# Autodesk Inventor assembly: Übertragung des Zahnriemens
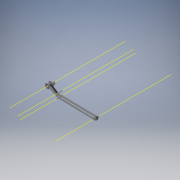
[picture p0: Inventor's stored thumbnail of the model, 180x180]
Saved by Autodesk Inventor 2019.1 (Build 231200000, 200)
## iProperties
Created: 2018-11-28
Part Number: Übertragung des Zahnriemens
Document SubType Name: Assembly
Designer: JochenAlt
ClientObjectVersion: 1
Author: JochenAlt
## Documents named in this file (6)
- D:\Projects\Ondine\CAD\Leg\LegInnerGear\Übertragung des Zahnriemens1.iam
- D:\Projects\Ondine\CAD\Leg\LegInnerGear\Zahnriemen1.ipt
- D:\Projects\Ondine\CAD\Leg\LegInnerGear\Synchrone Riemenscheibe11.ipt
- D:\Projects\Ondine\CAD\Leg\LegInnerGear\Synchrone Riemenscheibe21.ipt
- D:\Projects\Ondine\CAD\Leg\LegInnerGear\Flache Riemenscheibe11.ipt
- D:\Projects\Ondine\CAD\Leg\LegInnerGear\Synchrone Riemenscheibe31.ipt
## Components (5 placed, 5 different names)
1. Zahnriemen:1 — Fluchtend:1, Passend:1, Passend:2, Fluchtend:2, Passend:3, Passend:4, Fluchtend:3, Passend:5, Fluchtend:4, Passend:6, Passend:7
2. Synchrone Riemenscheibe1:1 — Fluchtend:1, Passend:1, Passend:2, Drehung:1, Drehung:2, Drehung:3
3. Synchrone Riemenscheibe2:1 — Fluchtend:2, Passend:3, Drehung:1, Passend:4
4. Flache Riemenscheibe1:1 — Fluchtend:3, Passend:5, Drehung:2
5. Synchrone Riemenscheibe3:1 — Fluchtend:4, Passend:6, Drehung:3, Passend:7
## Relationships (14: Mate 7, Flush 4, RelateRotation 3)
- Fluchtend:1 [Flush]: Zahnriemen:1 ↔ Synchrone Riemenscheibe1:1
- Passend:1 [Mate]: Zahnriemen:1 ↔ Synchrone Riemenscheibe1:1
- Passend:2 [Mate]: Zahnriemen:1 ↔ Synchrone Riemenscheibe1:1
- Fluchtend:2 [Flush]: Zahnriemen:1 ↔ Synchrone Riemenscheibe2:1
- Passend:3 [Mate]: Zahnriemen:1 ↔ Synchrone Riemenscheibe2:1
- Drehung:1 [RelateRotation] (1.6667 ul): Synchrone Riemenscheibe1:1 ↔ Synchrone Riemenscheibe2:1
- Passend:4 [Mate]: Zahnriemen:1 ↔ Synchrone Riemenscheibe2:1
- Fluchtend:3 [Flush] (-4.2 mm): Zahnriemen:1 ↔ Flache Riemenscheibe1:1
- Passend:5 [Mate]: Zahnriemen:1 ↔ Flache Riemenscheibe1:1
- Drehung:2 [RelateRotation] (0.5445 ul): Synchrone Riemenscheibe1:1 ↔ Flache Riemenscheibe1:1
- Fluchtend:4 [Flush]: Zahnriemen:1 ↔ Synchrone Riemenscheibe3:1
- Passend:6 [Mate]: Zahnriemen:1 ↔ Synchrone Riemenscheibe3:1
- Drehung:3 [RelateRotation] (1.6667 ul): Synchrone Riemenscheibe1:1 ↔ Synchrone Riemenscheibe3:1
- Passend:7 [Mate]: Zahnriemen:1 ↔ Synchrone Riemenscheibe3:1
